# Autodesk Inventor assembly: Cam crank
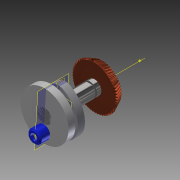
[picture p0: Inventor's stored thumbnail of the model, 180x180]
Saved by Autodesk Inventor 2015 (Build 190141000, 141)
## iProperties
Created: 2008-07-14
Part Number: Cam crank
Document SubType Name: Assembly
Designer: tangg
Mass: 210.119 g
Surface Area: 145.448 cm^2
Volume: 32.7179 cm^3
Density: 6.42214 g/cm^3
Author: tangg
## Documents named in this file (6)
- C:\Users\Aielloj\Downloads\inventor_2014_simulation\tutorial files\Dynamic Simulation 1 and 2\Cam crank.iam
- C:\Users\Aielloj\Downloads\inventor_2014_simulation\tutorial files\Dynamic Simulation 1 and 2\Crank shaft.ipt
- C:\Users\Aielloj\Downloads\inventor_2014_simulation\tutorial files\Dynamic Simulation 1 and 2\Roller.ipt
- C:\Users\Aielloj\Downloads\inventor_2014_simulation\tutorial files\Dynamic Simulation 1 and 2\Eccentric.ipt
- C:\Users\Aielloj\Downloads\inventor_2014_simulation\tutorial files\Dynamic Simulation 1 and 2\Bevel Gear21.ipt
- C:\Users\Aielloj\Downloads\inventor_2014_simulation\tutorial files\Dynamic Simulation 1 and 2\Cam  lobe.ipt
## Components (5 placed, 5 different names)
1. Crank shaft:1 — Flush:1, Mate:4, Mate:7, Mate:8, Flush:3, Mate:9
2. Roller:1 — Mate:2, Mate:3
3. Eccentric:1 — Mate:2, Mate:3, Flush:1, Mate:4, Mate:10
4. Bevel Gear2:1 — Mate:8, Flush:3
5. Cam  lobe:1 — Mate:9, Mate:10
## Relationships (9: Mate 7, Flush 2)
- Mate:2: Roller:1 ↔ Eccentric:1
- Mate:3: Roller:1 ↔ Eccentric:1
- Flush:1: Crank shaft:1 ↔ Eccentric:1
- Mate:4: Crank shaft:1 ↔ Eccentric:1
- Mate:7: Crank shaft:1
- Mate:8: Crank shaft:1 ↔ Bevel Gear2:1
- Flush:3 (-2.62 mm): Crank shaft:1 ↔ Bevel Gear2:1
- Mate:9: Crank shaft:1 ↔ Cam  lobe:1
- Mate:10: Eccentric:1 ↔ Cam  lobe:1
